# Autodesk Inventor assembly: VersaPlanetary Input MiniCIM v2
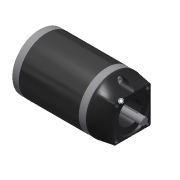
[picture p0: Inventor's stored thumbnail of the model, 180x180]
Saved by Autodesk Inventor 2015 (Build 190159000, 159)
## iProperties
Created: 2014-12-18
Part Number: VersaPlanetary Input MiniCIM v2
Document SubType Name: Assembly
Designer: Nemo
Author: Nemo
## Documents named in this file (4)
- H:\Nemo\Documents\Robotics\CAD Files\COTS Parts\Gearboxes\VersaPlanetary\VersaPlanetary Input MiniCIM v2.iam
- H:\Nemo\Documents\Robotics\CAD Files\COTS Parts\Gearboxes\VersaPlanetary\Components\VersaPlanetary CIM adapter.ipt
- H:\Nemo\Documents\Robotics\CAD Files\COTS Parts\Motors\Mini CIM.ipt
- H:\Nemo\Documents\Robotics\CAD Files\COTS Parts\Fasteners\10-32 SHCS x625.ipt
## Components (4 placed, 3 different names)
1. VersaPlanetary CIM adapter:1 — Mate:1, Mate:2, Flush:1, Mate:3, Mate:4, Mate:5, Insert:1, Insert:2
2. Mini CIM:1 — Mate:3, Mate:4, Mate:5
3. 10-32 SHCS x625:1 — Insert:1
4. 10-32 SHCS x625:2 — Insert:2
## Relationships (8: Mate 5, Insert 2, Flush 1)
- Mate:1: VersaPlanetary CIM adapter:1
- Mate:2: VersaPlanetary CIM adapter:1
- Flush:1: VersaPlanetary CIM adapter:1
- Mate:3: VersaPlanetary CIM adapter:1 ↔ Mini CIM:1
- Mate:4: VersaPlanetary CIM adapter:1 ↔ Mini CIM:1
- Mate:5: VersaPlanetary CIM adapter:1 ↔ Mini CIM:1
- Insert:1: VersaPlanetary CIM adapter:1 ↔ 10-32 SHCS x625:1
- Insert:2: VersaPlanetary CIM adapter:1 ↔ 10-32 SHCS x625:2
